# Autodesk Inventor assembly: OVA5647
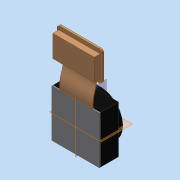
[picture p0: Inventor's stored thumbnail of the model, 180x180]
Saved by Autodesk Inventor 2016 SP1 (Build 200210100, 210)
## iProperties
Created: 2013-08-02
Part Number: OVA5647
Document SubType Name: Assembly
Designer: Mohamed A.
Sending System: SolidWorks 2014
Last Author: lavirott
Last Saved: 2015-02-19
Author: DFKI GmbH
Comments: http://www.dfki.de/robotik
## Documents named in this file (6)
- C:\Users\Mohamed\Documents\inventor\StemCellsPlatform\Camera\Raspberry Pi Camera rev 1.3\OVA5647.iam
- C:\Users\Mohamed\Documents\inventor\StemCellsPlatform\Camera\Raspberry Pi Camera rev 1.3\OVA5647.ipt
- C:\Users\Mohamed\Documents\inventor\StemCellsPlatform\Camera\Raspberry Pi Camera rev 1.3\OVA5647_Housing.ipt
- C:\Users\Mohamed\Documents\inventor\StemCellsPlatform\Camera\Raspberry Pi Camera rev 1.3\OVA5647_IR-Glas.ipt
- C:\Users\Mohamed\Documents\inventor\StemCellsPlatform\Camera\Raspberry Pi Camera rev 1.3\OVA5647_Lens.ipt
- C:\Users\Mohamed\Documents\inventor\StemCellsPlatform\Camera\Raspberry Pi Camera rev 1.3\OVA5647_Pigtail.ipt
## Components (5 placed, 5 different names)
1. OVA5647:1
2. OVA5647_Housing:1 — Angle:1, Angle:2
3. OVA5647_IR-Glas:1
4. OVA5647_Lens:1 — Mate:1, Mate:2
5. OVA5647_Pigtail:1
## Relationships (4: Mate 2, Angle 2)
- Mate:1: OVA5647_Lens:1
- Angle:1 (0 deg): OVA5647_Housing:1
- Mate:2: OVA5647_Lens:1
- Angle:2 (0 deg): OVA5647_Housing:1
